# Autodesk Inventor assembly: Arm
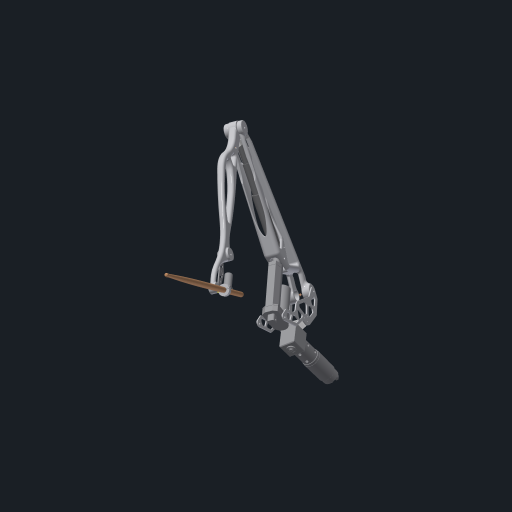
[picture p0: Inventor's stored thumbnail of the model, 512x512]
Saved by Autodesk Inventor 2023 (Build 270158000, 158)
## iProperties
Created: 2020-03-24
Part Number: Arm
Document SubType Name: Assembly
Designer: valer
Mass: 4853.13 g
Surface Area: 3141.52 cm^2
Volume: 1403.99 cm^3
Density: 3.45667 g/cm^3
Author: valer
## Documents named in this file (14)
- C:\Users\valer\Desktop\str1ker\cad\Arm.iam
- C:\Users\valer\Desktop\str1ker\cad\ArmBase.iam
- C:\Users\valer\Desktop\str1ker\cad\Shoulder.iam
- C:\Users\valer\Desktop\str1ker\cad\UpperArm.iam
- C:\Users\valer\Desktop\str1ker\cad\Forearm.iam
- C:\Users\valer\Desktop\str1ker\cad\Drumstick.iam
- C:\Users\valer\Desktop\str1ker\cad\ArmSolenoid.iam
- C:\Users\valer\Desktop\str1ker\cad\external\UpperArmActuator\UpperArmActuatorBase.iam
- C:\Users\valer\Desktop\str1ker\cad\external\UpperArmActuator\UpperArmActuatorShaft.iam
- C:\Users\valer\Desktop\str1ker\cad\external\ForearmActuator\ForearmActuatorBody.iam
- C:\Users\valer\Desktop\str1ker\cad\ForearmActuatorConnector.iam
- C:\Users\valer\Desktop\str1ker\cad\external\ForearmActuator\ForearmActuatorShaft.iam
- C:\Users\valer\Desktop\str1ker\cad\ArmBaseEncoderAlignmentFlange.ipt
- C:\Users\valer\Desktop\str1ker\cad\external\ArmEncoder\ArmEncoderShaftMagnet6mm.ipt
## Components (13 placed, 13 different names)
1. Base:1 [sub-assembly] — Mate:37, Mate:38, Mate:39, Mate:40, Mate:41
2. Shoulder:1 [sub-assembly] — Mate:4, Mate:5, Mate:26, Mate:27, Mate:37, Mate:38
3. UpperArm:1 [sub-assembly] — Mate:4, Mate:5, Mate:6, Mate:7, Mate:29, Flush:3, Mate:30
4. Forearm:1 [sub-assembly] — Mate:6, Mate:7, Mate:8, Mate:9, Mate:10, Mate:11, Mate:31
5. Drumstick:1 [sub-assembly] — Mate:8, Mate:9
6. ArmSolenoid:1 [sub-assembly] — Mate:10, Mate:11
7. UpperArmActuatorBase:1 [sub-assembly] — Mate:26, Mate:27, Mate:28
8. UpperArmActuatorShaft:1 [sub-assembly] — Mate:28, Mate:29
9. ForearmActuatorBody:1 [sub-assembly] — Flush:3, Mate:30, Mate:32, Mate:33
10. ForearmActuatorConnector:1 [sub-assembly] — Mate:31, Mate:32, Mate:34
11. ForearmActuatorShaft:1 [sub-assembly] — Mate:33, Mate:34
12. ArmBaseEncoderAlignmentFlange:1 — Mate:39, Flush:4
13. ArmEncoderShaftMagnet6mm:1 — Mate:40, Mate:41, Flush:4
## Relationships (24: Mate 22, Flush 2)
- Mate:4: Shoulder:1 ↔ UpperArm:1
- Mate:5: Shoulder:1 ↔ UpperArm:1
- Mate:6: UpperArm:1 ↔ Forearm:1
- Mate:7: UpperArm:1 ↔ Forearm:1
- Mate:8: Forearm:1 ↔ Drumstick:1
- Mate:9: Forearm:1 ↔ Drumstick:1
- Mate:10: Forearm:1 ↔ ArmSolenoid:1
- Mate:11: Forearm:1 ↔ ArmSolenoid:1
- Mate:26: Shoulder:1 ↔ UpperArmActuatorBase:1
- Mate:27: Shoulder:1 ↔ UpperArmActuatorBase:1
- Mate:28: UpperArmActuatorBase:1 ↔ UpperArmActuatorShaft:1
- Mate:29: UpperArm:1 ↔ UpperArmActuatorShaft:1
- Flush:3: UpperArm:1 ↔ ForearmActuatorBody:1
- Mate:30: UpperArm:1 ↔ ForearmActuatorBody:1
- Mate:31: Forearm:1 ↔ ForearmActuatorConnector:1
- Mate:32: ForearmActuatorBody:1 ↔ ForearmActuatorConnector:1
- Mate:33: ForearmActuatorBody:1 ↔ ForearmActuatorShaft:1
- Mate:34: ForearmActuatorConnector:1 ↔ ForearmActuatorShaft:1
- Mate:37: Base:1 ↔ Shoulder:1
- Mate:38: Base:1 ↔ Shoulder:1
- Mate:39: Base:1 ↔ ArmBaseEncoderAlignmentFlange:1
- Mate:40: Base:1 ↔ ArmEncoderShaftMagnet6mm:1
- Mate:41: Base:1 ↔ ArmEncoderShaftMagnet6mm:1
- Flush:4: ArmBaseEncoderAlignmentFlange:1 ↔ ArmEncoderShaftMagnet6mm:1
